# Autodesk Inventor assembly: J005658
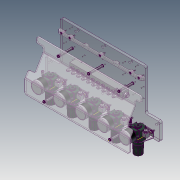
[picture p0: Inventor's stored thumbnail of the model, 180x180]
Saved by Autodesk Inventor 2015 SP1 (Build 190203100, 203)
## iProperties
Created: 2015-05-14
Vendor: HHMI: JRC - ID&F
Document SubType Name: Assembly
Designer: ARNOLDJ
Part Number: J005658
Description: MBS REGULATOR AND MANIFOLD ASSY
RuleStatus: InUse
AfterDocSave0: file://Part Number Cleaner
DESIGN DEPARTMENT: HHMI: JRC - ID&F
ALTERED ITEM PART NUMBER: N/A
ALTERED ITEM VENDOR: N/A
ALTERED ITEM DESCRIPTION: N/A
Revision Number: 0
## Documents named in this file (16)
- C:\_WORKSPACE\DATA\COLLABORATION\SVOBODA LAB\MOUSE POSITIONING SYSTEMS\MCAD\BALL SETUP\MBS REG AND MANIFOLD PLATE ASSY.iam
- C:\_WORKSPACE\DATA\COLLABORATION\SVOBODA LAB\MOUSE POSITIONING SYSTEMS\MCAD\BALL SETUP\MBS REG BASE PLATE.ipt
- C:\_WORKSPACE\DATA\COLLABORATION\SVOBODA LAB\MOUSE POSITIONING SYSTEMS\MCAD\BALL SETUP\MBS REGULATOR ASSY.iam
- C:\_WORKSPACE\DATA\COLLABORATION\SVOBODA LAB\MOUSE POSITIONING SYSTEMS\MCAD\BALL SETUP\5085K910.ipt
- C:\_WORKSPACE\DATA\COLLABORATION\SVOBODA LAB\MOUSE POSITIONING SYSTEMS\MCAD\BALL SETUP\5779K143.ipt
- C:\_WORKSPACE\DATA\COLLABORATION\SVOBODA LAB\MOUSE POSITIONING SYSTEMS\MCAD\BALL SETUP\95947A074.ipt
- C:\_WORKSPACE\DATA\COLLABORATION\SVOBODA LAB\MOUSE POSITIONING SYSTEMS\MCAD\BALL SETUP\MBS DEFLECTOR SHIELD .ipt
- C:\_WORKSPACE\DATA\COLLABORATION\SVOBODA LAB\MOUSE POSITIONING SYSTEMS\MCAD\BALL SETUP\MBS TROUGH RAIL.ipt
- C:\_WORKSPACE\DATA\COLLABORATION\SVOBODA LAB\MOUSE POSITIONING SYSTEMS\MCAD\BALL SETUP\93475A240.ipt
- C:\_WORKSPACE\DATA\COLLABORATION\SVOBODA LAB\MOUSE POSITIONING SYSTEMS\MCAD\BALL SETUP\92000A320.ipt
- C:\_WORKSPACE\DATA\COLLABORATION\SVOBODA LAB\MOUSE POSITIONING SYSTEMS\MCAD\BALL SETUP\92010A226.ipt
- C:\_WORKSPACE\DATA\COLLABORATION\SVOBODA LAB\MOUSE POSITIONING SYSTEMS\MCAD\BALL SETUP\93475A230.ipt
- C:\_WORKSPACE\DATA\COLLABORATION\SVOBODA LAB\MOUSE POSITIONING SYSTEMS\MCAD\BALL SETUP\90116A207.ipt
- C:\_WORKSPACE\DATA\COLLABORATION\SVOBODA LAB\MOUSE POSITIONING SYSTEMS\MCAD\BALL SETUP\50785K213.ipt
- C:\_WORKSPACE\DATA\COLLABORATION\SVOBODA LAB\MOUSE POSITIONING SYSTEMS\MCAD\BALL SETUP\5779K109.ipt
- C:\_WORKSPACE\DATA\COLLABORATION\SVOBODA LAB\MOUSE POSITIONING SYSTEMS\MCAD\BALL SETUP\92000A234.ipt
## Components (75 placed, 15 different names)
1. MBS REG BASE PLATE:1 — Mate:1, Mate:2, Mate:3, Mate:4, Mate:5, Mate:6, Mate:10, Mate:11, Mate:16, Mate:17, Mate:18, Mate:19, Mate:20, Mate:21, Mate:22, Mate:23, Mate:26, Mate:27, Mate:28, Mate:30, Mate:32, Mate:42, Mate:43, Mate:44, Mate:45, Mate:46, Mate:47, Mate:48, Mate:49, Mate:50, Mate:51
2. 5085K910:1 — Mate:4, Mate:5, Mate:6, Mate:7, Mate:8, Mate:9, Flush:6, Mate:82, Mate:83, Mate:84, Mate:85, Mate:86, Mate:87, Mate:88
3. 95947A074:1 — Mate:10, Mate:11, Mate:12, Mate:13
4. 95947A074:2 — Mate:12, Mate:13, Mate:14, Mate:15, Mate:58, Mate:59
5. MBS DEFLECTOR SHIELD :1 — Mate:14, Mate:15, Mate:62, Mate:64, Mate:66, Mate:68, Mate:69, Mate:70
6. 95947A074:3 — Mate:22, Mate:23, Mate:24, Mate:25
7. 95947A074:4 — Mate:24, Mate:25, Mate:60, Mate:61, Mate:71
8. 95947A074:5 — Mate:20, Mate:21, Mate:52, Mate:53
9. 95947A074:6 — Mate:18, Mate:19, Mate:54, Mate:55, Mate:65
10. 95947A074:7 — Mate:16, Mate:17, Mate:56, Mate:57, Mate:67
11. MBS TROUGH RAIL:1 — Mate:26, Mate:27, Mate:28, Flush:1, Mate:37, Flush:2, Mate:38, Flush:3, Mate:39, Mate:40, Flush:4, Mate:41, Flush:5
12. 92010A226:1 — Flush:1, Mate:37
13. 92010A226:2 — Flush:2, Mate:38
14. 92010A226:3 — Flush:3, Mate:39
15. 92010A226:4 — Mate:40, Flush:4
16. 92010A226:5 — Mate:41, Flush:5
17. 93475A230:1 — Mate:50, Mate:51
18. 93475A230:2 — Mate:48, Mate:49
19. 93475A230:3 — Mate:42, Mate:43
20. 93475A230:4 — Mate:44, Mate:45
21. 93475A230:5 — Mate:46, Mate:47
22. 93475A230:6 — Mate:52, Mate:53, Mate:63
23. 93475A230:7 — Mate:54, Mate:55
24. 93475A230:8 — Mate:56, Mate:57
25. 93475A230:9 — Mate:58, Mate:59
26. 93475A230:10 — Mate:60, Mate:61
27. 93475A230:11 — Mate:70, Mate:71, Mate:80, Mate:81
28. 93475A230:12 — Mate:68, Mate:69, Mate:78, Mate:79
29. 93475A230:13 — Mate:66, Mate:67, Mate:76, Mate:77
30. 93475A230:14 — Mate:64, Mate:65, Mate:74, Mate:75
31. 93475A230:15 — Mate:62, Mate:63, Mate:72, Mate:73
32. 90116A207:1 — Mate:80, Mate:81
33. 90116A207:2 — Mate:78, Mate:79
34. 90116A207:3 — Mate:76, Mate:77
35. 90116A207:4 — Mate:74, Mate:75
36. 90116A207:5 — Mate:72, Mate:73
37. 50785K213:1 — Flush:6, Mate:82
38. 5779K109:1 — Mate:83, Mate:84
39. 92000A234:1 — Mate:87, Mate:88
40. 92000A234:2 — Mate:85, Mate:86
41. MBS REGULATOR ASSY:1 [sub-assembly] — Mate:1, Mate:2, Mate:3, Mate:29, Mate:31
42. MBS REGULATOR ASSY:2 [sub-assembly]
43. MBS REGULATOR ASSY:3 [sub-assembly]
44. MBS REGULATOR ASSY:4 [sub-assembly]
45. MBS REGULATOR ASSY:5 [sub-assembly]
46. 92000A320:2 — Mate:35, Mate:36
47. 92000A320:1 — Mate:33, Mate:34
48. 93475A240:2 — Mate:31, Mate:32, Mate:35, Mate:36
49. 93475A240:1 — Mate:29, Mate:30, Mate:33, Mate:34
50. 92000A320:3
51. 92000A320:4
52. 93475A240:3
53. 93475A240:4
54. 92000A320:5
55. 92000A320:6
56. 93475A240:5
57. 93475A240:6
58. 92000A320:7
59. 92000A320:8
60. 93475A240:7
61. 93475A240:8
62. 92000A320:9
63. 92000A320:10
64. 93475A240:9
65. 93475A240:10
66. 5779K143:1 — Mate:7, Mate:8, Mate:9
67. 5779K143:2
68. 5779K143:3
69. 5779K143:4
70. 5779K143:5
71. 5779K143:6
72. 5779K143:7
73. 5779K143:8
74. 5779K143:9
75. 5779K143:10
## Component patterns: (5 elements, first: MBS REGULATOR ASSY:1), (5 elements, first: 92000A320:2 + 92000A320:1 + 93475A240:2 + 93475A240:1), (10 elements, first: 5779K143:1)
## Relationships (94: Mate 88, Flush 6)
- Mate:1: MBS REG BASE PLATE:1 ↔ MBS REGULATOR ASSY:1
- Mate:2: MBS REG BASE PLATE:1 ↔ MBS REGULATOR ASSY:1
- Mate:3: MBS REG BASE PLATE:1 ↔ MBS REGULATOR ASSY:1
- Mate:4: MBS REG BASE PLATE:1 ↔ 5085K910:1
- Mate:5: MBS REG BASE PLATE:1 ↔ 5085K910:1
- Mate:6: MBS REG BASE PLATE:1 ↔ 5085K910:1
- Mate:7 (1.27 mm): 5085K910:1 ↔ 5779K143:1
- Mate:8 (1.27 mm): 5085K910:1 ↔ 5779K143:1
- Mate:9: 5085K910:1 ↔ 5779K143:1
- Mate:10: MBS REG BASE PLATE:1 ↔ 95947A074:1
- Mate:11 (0.889 mm): MBS REG BASE PLATE:1 ↔ 95947A074:1
- Mate:12: 95947A074:1 ↔ 95947A074:2
- Mate:13: 95947A074:1 ↔ 95947A074:2
- Mate:14 (0.889 mm): 95947A074:2 ↔ MBS DEFLECTOR SHIELD :1
- Mate:15: 95947A074:2 ↔ MBS DEFLECTOR SHIELD :1
- Mate:16: MBS REG BASE PLATE:1 ↔ 95947A074:7
- Mate:17 (0.889 mm): MBS REG BASE PLATE:1 ↔ 95947A074:7
- Mate:18 (0.889 mm): MBS REG BASE PLATE:1 ↔ 95947A074:6
- Mate:19: MBS REG BASE PLATE:1 ↔ 95947A074:6
- Mate:20 (0.889 mm): MBS REG BASE PLATE:1 ↔ 95947A074:5
- Mate:21: MBS REG BASE PLATE:1 ↔ 95947A074:5
- Mate:22: MBS REG BASE PLATE:1 ↔ 95947A074:3
- Mate:23 (0.889 mm): MBS REG BASE PLATE:1 ↔ 95947A074:3
- Mate:24: 95947A074:3 ↔ 95947A074:4
- Mate:25: 95947A074:3 ↔ 95947A074:4
- Mate:26: MBS REG BASE PLATE:1 ↔ MBS TROUGH RAIL:1
- Mate:27: MBS REG BASE PLATE:1 ↔ MBS TROUGH RAIL:1
- Mate:28: MBS REG BASE PLATE:1 ↔ MBS TROUGH RAIL:1
- Mate:29: MBS REGULATOR ASSY:1 ↔ 93475A240:1
- Mate:30: MBS REG BASE PLATE:1 ↔ 93475A240:1
- Mate:31: MBS REGULATOR ASSY:1 ↔ 93475A240:2
- Mate:32: MBS REG BASE PLATE:1 ↔ 93475A240:2
- Mate:33: 92000A320:1 ↔ 93475A240:1
- Mate:34: 92000A320:1 ↔ 93475A240:1
- Mate:35: 92000A320:2 ↔ 93475A240:2
- Mate:36: 92000A320:2 ↔ 93475A240:2
- Flush:1 (0.508 mm): MBS TROUGH RAIL:1 ↔ 92010A226:1
- Mate:37: MBS TROUGH RAIL:1 ↔ 92010A226:1
- Flush:2 (0.508 mm): MBS TROUGH RAIL:1 ↔ 92010A226:2
- Mate:38: MBS TROUGH RAIL:1 ↔ 92010A226:2
- Flush:3 (0.508 mm): MBS TROUGH RAIL:1 ↔ 92010A226:3
- Mate:39: MBS TROUGH RAIL:1 ↔ 92010A226:3
- Mate:40: MBS TROUGH RAIL:1 ↔ 92010A226:4
- Flush:4 (0.508 mm): MBS TROUGH RAIL:1 ↔ 92010A226:4
- Mate:41: MBS TROUGH RAIL:1 ↔ 92010A226:5
- Flush:5 (0.508 mm): MBS TROUGH RAIL:1 ↔ 92010A226:5
- Mate:42: MBS REG BASE PLATE:1 ↔ 93475A230:3
- Mate:43: MBS REG BASE PLATE:1 ↔ 93475A230:3
- Mate:44: MBS REG BASE PLATE:1 ↔ 93475A230:4
- Mate:45: MBS REG BASE PLATE:1 ↔ 93475A230:4
- Mate:46: MBS REG BASE PLATE:1 ↔ 93475A230:5
- Mate:47: MBS REG BASE PLATE:1 ↔ 93475A230:5
- Mate:48: MBS REG BASE PLATE:1 ↔ 93475A230:2
- Mate:49: MBS REG BASE PLATE:1 ↔ 93475A230:2
- Mate:50: MBS REG BASE PLATE:1 ↔ 93475A230:1
- Mate:51: MBS REG BASE PLATE:1 ↔ 93475A230:1
- Mate:52: 95947A074:5 ↔ 93475A230:6
- Mate:53: 95947A074:5 ↔ 93475A230:6
- Mate:54: 95947A074:6 ↔ 93475A230:7
- Mate:55: 95947A074:6 ↔ 93475A230:7
- Mate:56: 95947A074:7 ↔ 93475A230:8
- Mate:57: 95947A074:7 ↔ 93475A230:8
- Mate:58: 95947A074:2 ↔ 93475A230:9
- Mate:59: 95947A074:2 ↔ 93475A230:9
- Mate:60: 95947A074:4 ↔ 93475A230:10
- Mate:61: 95947A074:4 ↔ 93475A230:10
- Mate:62: MBS DEFLECTOR SHIELD :1 ↔ 93475A230:15
- Mate:63: 93475A230:6 ↔ 93475A230:15
- Mate:64: MBS DEFLECTOR SHIELD :1 ↔ 93475A230:14
- Mate:65: 95947A074:6 ↔ 93475A230:14
- Mate:66: MBS DEFLECTOR SHIELD :1 ↔ 93475A230:13
- Mate:67: 95947A074:7 ↔ 93475A230:13
- Mate:68: MBS DEFLECTOR SHIELD :1 ↔ 93475A230:12
- Mate:69: MBS DEFLECTOR SHIELD :1 ↔ 93475A230:12
- Mate:70: MBS DEFLECTOR SHIELD :1 ↔ 93475A230:11
- Mate:71: 95947A074:4 ↔ 93475A230:11
- Mate:72: 93475A230:15 ↔ 90116A207:5
- Mate:73: 93475A230:15 ↔ 90116A207:5
- Mate:74: 93475A230:14 ↔ 90116A207:4
- Mate:75: 93475A230:14 ↔ 90116A207:4
- Mate:76: 93475A230:13 ↔ 90116A207:3
- Mate:77: 93475A230:13 ↔ 90116A207:3
- Mate:78: 93475A230:12 ↔ 90116A207:2
- Mate:79: 93475A230:12 ↔ 90116A207:2
- Mate:80: 93475A230:11 ↔ 90116A207:1
- Mate:81: 93475A230:11 ↔ 90116A207:1
- Flush:6: 5085K910:1 ↔ 50785K213:1
- Mate:82: 5085K910:1 ↔ 50785K213:1
- Mate:83 (1.27 mm): 5085K910:1 ↔ 5779K109:1
- Mate:84: 5085K910:1 ↔ 5779K109:1
- Mate:85: 5085K910:1 ↔ 92000A234:2
- Mate:86: 5085K910:1 ↔ 92000A234:2
- Mate:87: 5085K910:1 ↔ 92000A234:1
- Mate:88: 5085K910:1 ↔ 92000A234:1
